# Autodesk Inventor assembly: ASY MSC 100.2 CONE TUBE
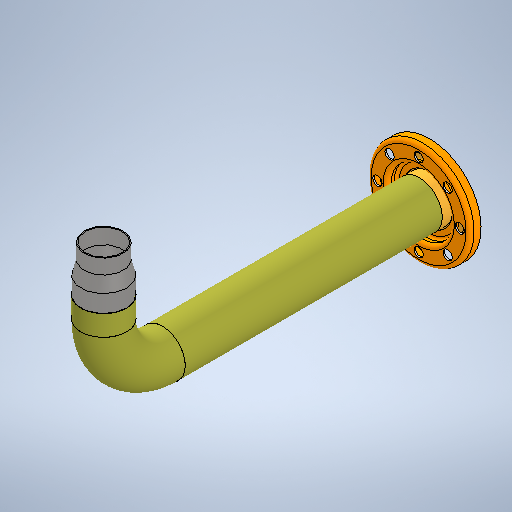
[picture p0: Inventor's stored thumbnail of the model, 512x512]
Saved by Autodesk Inventor 2025.1 (Build 291241020, 241B)
## iProperties
Created: 2024-08-28
Part Number: ASY MSC 100.2 CONE TUBE
Document SubType Name: Assembly
Designer: admin
Stock Number: ASY МОО 100.2 конус труба
Author: admin
## Documents named in this file (7)
- C:\Users\user\YandexDisk-badmisterfox\домашниий пк\Inventor\Manturovo\Manturovo_Se-clar\ASY MSC 100.2 Cone tube.iam
- C:\Users\user\YandexDisk-badmisterfox\домашниий пк\Inventor\Manturovo\Manturovo_Se-clar\MSC 104 tube.ipt
- C:\Users\user\YandexDisk-badmisterfox\домашниий пк\Inventor\Manturovo\Manturovo_Se-clar\MSC 105 rocket tube 9.ipt
- C:\Users\user\YandexDisk-badmisterfox\домашниий пк\Inventor\Manturovo\Manturovo_Se-clar\JIS B 2312 Concentric Reducer Stainless Steel 80A x 65A x Sch5S.ipt
- C:\Users\user\YandexDisk-badmisterfox\домашниий пк\Inventor\Manturovo\Manturovo_Se-clar\ISO 5251 Bends 3D without straight ends(90 deg) DN80 2 2.ipt
- C:\Users\user\YandexDisk-badmisterfox\домашниий пк\Inventor\Manturovo\Manturovo_Se-clar\3d party\Stamp flange DIN2642\Stamd flange lapped collar DIN2642\Stamp flange DIN2642-080.ipt
- C:\Users\pokla\Documents\Inventor\Отстойник осветлитель\Manturovo_Se-clar-Gleb\Stamd flange lapped collar DIN2642.ipt
## Components (5 placed, 5 different names)
1. MSC 104 tube.ipt:1 — Rigid:2, Rigid:4
2. MSC 105 rocket tube 9.ipt:1 — Rigid:3
3. JIS B 2312 Concentric Reducer Stainless Steel 80A x 65A x Sch5S.ipt:1
4. ISO 5251 Bends 3D without straight ends(90 deg) DN80 2 2.ipt:1 — Rigid:2, Rigid:3
5. Stamp flange DIN2642-080.ipt:1 — Rigid:4
## Relationships (4: WeldJoint 3, RevoluteJoint 1)
- [RevoluteJoint]: MSC 105 rocket tube 9.ipt:1 ↔ JIS B 2312 Concentric Reducer Stainless Steel 80A x 65A x Sch5S.ipt:1
- Rigid:2 [WeldJoint]: MSC 104 tube.ipt:1 ↔ ISO 5251 Bends 3D without straight ends(90 deg) DN80 2 2.ipt:1
- Rigid:3 [WeldJoint]: MSC 105 rocket tube 9.ipt:1 ↔ ISO 5251 Bends 3D without straight ends(90 deg) DN80 2 2.ipt:1
- Rigid:4 [WeldJoint]: MSC 104 tube.ipt:1 ↔ Stamp flange DIN2642-080.ipt:1
